# Autodesk Inventor assembly: Switch AV4524
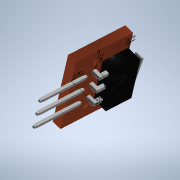
[picture p0: Inventor's stored thumbnail of the model, 180x180]
Saved by Autodesk Inventor 2020.3 (Build 243373000, 373)
## iProperties
Created: 2020-06-09
Part Number: Switch AV4524
Document SubType Name: Assembly
Designer: javic
Author: javic
## Documents named in this file (4)
- C:\Users\javic\Downloads\Universidad\2020-1\Seminario - SPEL\InterStage\Componentes\Piezas\Switch AV4524.iam
- C:\Users\javic\Downloads\Universidad\2020-1\Seminario - SPEL\InterStage\Componentes\Piezas\Placa Cobre.ipt
- C:\Users\javic\Downloads\Universidad\2020-1\Seminario - SPEL\InterStage\Componentes\Piezas\Switch AV4524.ipt
- C:\Users\javic\Downloads\Universidad\2020-1\Seminario - SPEL\InterStage\Componentes\Piezas\Conector 3 pines.ipt
## Components (3 placed, 3 different names)
1. Placa Cobre:1 — Coincidencia:68, Nivelación:38, Coincidencia:70, Coincidencia:81
2. Switch AV4524:1 — Coincidencia:68, Nivelación:38, Coincidencia:71, Nivelación:39, Coincidencia:81
3. Conector 3 pines:1 — Coincidencia:70, Coincidencia:71, Nivelación:39
## Relationships (6: Mate 4, Flush 2)
- Coincidencia:68 [Mate]: Placa Cobre:1 ↔ Switch AV4524:1
- Nivelación:38 [Flush] (2.75 mm): Placa Cobre:1 ↔ Switch AV4524:1
- Coincidencia:70 [Mate]: Placa Cobre:1 ↔ Conector 3 pines:1
- Coincidencia:71 [Mate] (1.17 mm): Switch AV4524:1 ↔ Conector 3 pines:1
- Nivelación:39 [Flush] (0.05 mm): Switch AV4524:1 ↔ Conector 3 pines:1
- Coincidencia:81 [Mate]: Placa Cobre:1 ↔ Switch AV4524:1
